# Autodesk Inventor assembly: Uchwyt_konwerter
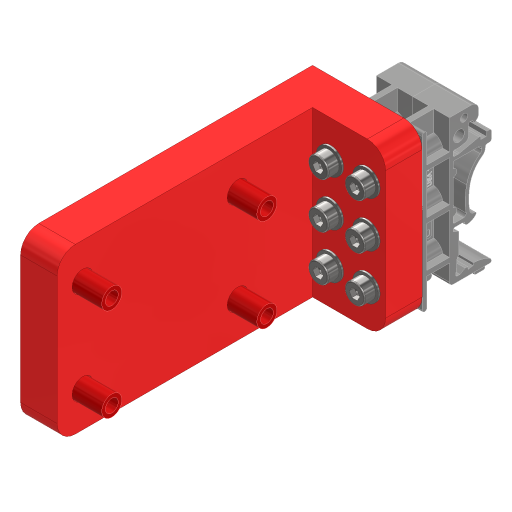
[picture p0: Inventor's stored thumbnail of the model, 512x512]
Saved by Autodesk Inventor 2024.3 (Build 283343000, 343)
## iProperties
Created: 2025-06-30
Part Number: Uchwyt_konwerter
Document SubType Name: Assembly
Designer: PM
Author: PM
## Documents named in this file (6)
- C:\MPA - shortPath\magisterka\V3\Workspace\MontazWszafie\Uchwyt_konwerter.iam
- C:\MPA - shortPath\magisterka\V3\Workspace\MontazWszafie\Uchwyt_konwerter.ipt
- C:\MPA - shortPath\magisterka\V3\Workspace\MontazWszafie\Arduino-cz2.ipt
- C:\MPA - shortPath\magisterka\V3\Workspace\MontazWszafie\1201578_PHOENIX\1201578_PHOENIX\1201578_PHOENIX.ipt
- C:\MPA - shortPath\magisterka\V3\Workspace\cc\en-US\DIN 125-1  A\DIN 125 - A 3,2.ipt
- C:\MPA - shortPath\magisterka\V3\Workspace\cc\en-US\Copy of DIN 912 - replaced by DIN EN ISO 4762\Copy of DIN 912 - M3 x 0,5 x 16 x 14,75.ipt
## Components (19 placed, 5 different names)
1. Uchwyt_konwerter:1 — Flush:1, Flush:2, Flush:3, Insert:1, Insert:2, Mate:1, Mate:2, Insert:3, Insert:4, Insert:5, Insert:6, Mate:3, Mate:4, Mate:5, Mate:6, Mate:7, Mate:8, Mate:9, Mate:10, Mate:11, Mate:12, Mate:13, Mate:14
2. Arduino-cz2:1 — Insert:3
3. 1201578_PHOENIX:1 — Insert:2, Mate:1
4. 1201578_PHOENIX:2 — Insert:1, Mate:2
5. Arduino-cz2:2 — Insert:4
6. Arduino-cz2:3 — Insert:5
7. Arduino-cz2:4 — Insert:6
8. DIN 125-1 A A 3,2:1 — Mate:3, Mate:4, Insert:7
9. Copy of DIN 912 - replaced by DIN EN ISO 4762 M3 x 16:1 — Insert:7
10. DIN 125-1 A A 3,2:2 — Mate:5, Mate:6, Insert:8
11. DIN 125-1 A A 3,2:3 — Mate:7, Mate:8, Insert:9
12. DIN 125-1 A A 3,2:4 — Mate:9, Mate:10, Insert:10
13. DIN 125-1 A A 3,2:5 — Mate:11, Mate:12, Insert:11
14. DIN 125-1 A A 3,2:6 — Mate:13, Mate:14, Insert:12
15. Copy of DIN 912 - replaced by DIN EN ISO 4762 M3 x 16:2 — Insert:8
16. Copy of DIN 912 - replaced by DIN EN ISO 4762 M3 x 16:3 — Insert:9
17. Copy of DIN 912 - replaced by DIN EN ISO 4762 M3 x 16:4 — Insert:10
18. Copy of DIN 912 - replaced by DIN EN ISO 4762 M3 x 16:5 — Insert:11
19. Copy of DIN 912 - replaced by DIN EN ISO 4762 M3 x 16:6 — Insert:12
## Relationships (29: Mate 14, Insert 12, Flush 3)
- Flush:1: Uchwyt_konwerter:1
- Flush:2: Uchwyt_konwerter:1
- Flush:3: Uchwyt_konwerter:1
- Insert:1: Uchwyt_konwerter:1 ↔ 1201578_PHOENIX:2
- Insert:2: Uchwyt_konwerter:1 ↔ 1201578_PHOENIX:1
- Mate:1: Uchwyt_konwerter:1 ↔ 1201578_PHOENIX:1
- Mate:2: Uchwyt_konwerter:1 ↔ 1201578_PHOENIX:2
- Insert:3: Uchwyt_konwerter:1 ↔ Arduino-cz2:1
- Insert:4: Uchwyt_konwerter:1 ↔ Arduino-cz2:2
- Insert:5: Uchwyt_konwerter:1 ↔ Arduino-cz2:3
- Insert:6: Uchwyt_konwerter:1 ↔ Arduino-cz2:4
- Mate:3: Uchwyt_konwerter:1 ↔ DIN 125-1 A A 3,2:1
- Mate:4: Uchwyt_konwerter:1 ↔ DIN 125-1 A A 3,2:1
- Mate:5: Uchwyt_konwerter:1 ↔ DIN 125-1 A A 3,2:2
- Mate:6: Uchwyt_konwerter:1 ↔ DIN 125-1 A A 3,2:2
- Mate:7: Uchwyt_konwerter:1 ↔ DIN 125-1 A A 3,2:3
- Mate:8: Uchwyt_konwerter:1 ↔ DIN 125-1 A A 3,2:3
- Mate:9: Uchwyt_konwerter:1 ↔ DIN 125-1 A A 3,2:4
- Mate:10: Uchwyt_konwerter:1 ↔ DIN 125-1 A A 3,2:4
- Mate:11: Uchwyt_konwerter:1 ↔ DIN 125-1 A A 3,2:5
- Mate:12: Uchwyt_konwerter:1 ↔ DIN 125-1 A A 3,2:5
- Mate:13: Uchwyt_konwerter:1 ↔ DIN 125-1 A A 3,2:6
- Mate:14: Uchwyt_konwerter:1 ↔ DIN 125-1 A A 3,2:6
- Insert:7: DIN 125-1 A A 3,2:1 ↔ Copy of DIN 912 - replaced by DIN EN ISO 4762 M3 x 16:1
- Insert:8: DIN 125-1 A A 3,2:2 ↔ Copy of DIN 912 - replaced by DIN EN ISO 4762 M3 x 16:2
- Insert:9: DIN 125-1 A A 3,2:3 ↔ Copy of DIN 912 - replaced by DIN EN ISO 4762 M3 x 16:3
- Insert:10: DIN 125-1 A A 3,2:4 ↔ Copy of DIN 912 - replaced by DIN EN ISO 4762 M3 x 16:4
- Insert:11: DIN 125-1 A A 3,2:5 ↔ Copy of DIN 912 - replaced by DIN EN ISO 4762 M3 x 16:5
- Insert:12: DIN 125-1 A A 3,2:6 ↔ Copy of DIN 912 - replaced by DIN EN ISO 4762 M3 x 16:6
